# Autodesk Inventor assembly: FullEnd
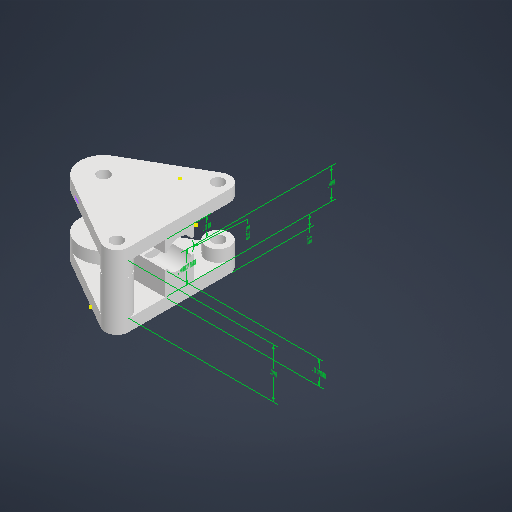
[picture p0: Inventor's stored thumbnail of the model, 512x512]
Saved by Autodesk Inventor 2026 (Build 300175000, 175)
## iProperties
Created: 2025-04-10
Part Number: FullEnd
Document SubType Name: Assembly
Designer: jjgen
Author: jjgen
## Documents named in this file (3)
- C:\Users\jjgen\OneDrive\Documents\Inventor\Curtain Opener\FullEnd.iam
- C:\Users\jjgen\OneDrive\Documents\Inventor\Curtain Opener\End.ipt
- C:\Users\jjgen\OneDrive\Documents\Inventor\Curtain Opener\EndTop3.ipt
## Components (2 placed, 2 different names)
1. End:1 — Mate:1
2. EndTop3:1 — Mate:1
## Relationships (1: Mate 1)
- Mate:1: End:1 ↔ EndTop3:1
